# Autodesk Inventor assembly: Cartridge Assembly Exploded
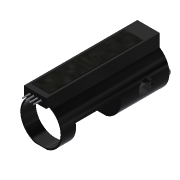
[picture p0: Inventor's stored thumbnail of the model, 180x180]
Saved by Autodesk Inventor 2017 (Build 210142000, 142)
## iProperties
Created: 2017-01-02
Part Number: Cartridge Assembly Exploded
Document SubType Name: Assembly
Designer: ge937963
Author: ge937963
## Documents named in this file (8)
- C:\Users\ge937963\Desktop\Inventor View\Cartridge.iam
- C:\Users\ge937963\Desktop\Inventor View\Cartridge Housing.ipt
- C:\Users\ge937963\Desktop\Inventor View\Heater Holder.ipt
- C:\Users\ge937963\Desktop\Inventor View\Screw.ipt
- C:\Users\ge937963\Desktop\Inventor View\PCR Tube.ipt
- C:\Users\ge937963\Desktop\Inventor View\Heating Block.iam
- C:\Users\ge937963\Desktop\Inventor View\Wire Cover.ipt
- C:\Users\ge937963\Desktop\Inventor View\4 Pin Male.iam
## Components (9 placed, 7 different names)
1. Cartridge Housing:1 — Mate:1, Flush:1, Mate:2, Flush:2, Mate:7, Mate:9, Mate:10, Mate:11, Mate:12, Mate:13, Flush:5, Angle:1, Mate:16, Mate:17
2. Heater Holder:1 — Mate:1, Flush:1, Mate:4, Mate:5, Mate:6, Mate:8, Mate:13, Mate:14, Mate:15
3. Screw:1 — Mate:4, Flush:3, Flush:4, Mate:14
4. Screw:2 — Mate:6, Flush:4
5. Screw:3 — Mate:5, Flush:3
6. PCR Tube:1 — Mate:7, Mate:16
7. Heating Block:1 [sub-assembly] — Mate:8, Mate:15, Angle:1
8. Wire Cover:1 — Mate:9, Mate:10, Flush:5
9. 4 Pin Male:1 [sub-assembly] — Mate:11, Mate:12, Mate:17
## Relationships (22: Mate 16, Flush 5, Angle 1)
- Mate:1: Cartridge Housing:1 ↔ Heater Holder:1
- Flush:1: Cartridge Housing:1 ↔ Heater Holder:1
- Mate:2: Cartridge Housing:1
- Flush:2: Cartridge Housing:1
- Mate:4: Heater Holder:1 ↔ Screw:1
- Mate:5: Heater Holder:1 ↔ Screw:3
- Mate:6: Heater Holder:1 ↔ Screw:2
- Flush:3: Screw:1 ↔ Screw:3
- Flush:4: Screw:1 ↔ Screw:2
- Mate:7: Cartridge Housing:1 ↔ PCR Tube:1
- Mate:8: Heater Holder:1 ↔ Heating Block:1
- Mate:9 (0.508 mm): Cartridge Housing:1 ↔ Wire Cover:1
- Mate:10 (0.508 mm): Cartridge Housing:1 ↔ Wire Cover:1
- Mate:11: Cartridge Housing:1 ↔ 4 Pin Male:1
- Mate:12: Cartridge Housing:1 ↔ 4 Pin Male:1
- Mate:13: Cartridge Housing:1 ↔ Heater Holder:1
- Mate:14: Heater Holder:1 ↔ Screw:1
- Flush:5: Cartridge Housing:1 ↔ Wire Cover:1
- Mate:15: Heater Holder:1 ↔ Heating Block:1
- Angle:1 (0 deg): Cartridge Housing:1 ↔ Heating Block:1
- Mate:16: Cartridge Housing:1 ↔ PCR Tube:1
- Mate:17: Cartridge Housing:1 ↔ 4 Pin Male:1
